# Autodesk Inventor assembly: rigt_motor_asembly
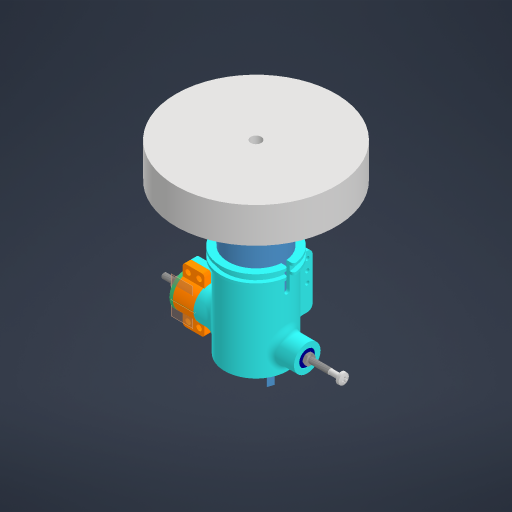
[picture p0: Inventor's stored thumbnail of the model, 512x512]
Saved by Autodesk Inventor 2024 (Build 280153000, 153)
## iProperties
Created: 2023-05-14
Part Number: rigt_motor_asembly
Document SubType Name: Assembly
Designer: user
Author: user
## Documents named in this file (9)
- D:\Docs\Robot\3d\motor_assembly\left_motor_asembly.iam
- D:\Docs\Robot\3d\motor_assembly\bushing_assembly.iam
- D:\Docs\Robot\3d\default_components\motor.ipt
- D:\Docs\Robot\3d\default_components\wheel.ipt
- D:\Docs\Robot\3d\default_components\604zz_bearing.ipt
- C:\Users\user\Documents\Inventor\Content Center Files\R2024\ru-RU\DIN 934\DIN 934 - M4 x 0,7.ipt
- D:\Docs\Robot\3d\motor_assembly\default_motor_asembly\cup.ipt
- D:\Docs\Robot\3d\motor_assembly\left_motor_asembly\lower_arm.ipt
- C:\Users\user\Documents\Inventor\Content Center Files\R2024\ru-RU\DIN 7985 (H)\DIN 7985 (H) - M4x30-H.ipt
## Components (8 placed, 8 different names)
1. lower_arm:2 — Вставка:11, Вставка:12, Вставка:13, Вставка:14, Вставка:15
2. bushing_assembly:2 [sub-assembly] — Вставка:14
3. motor:1 — Вставка:4, Вставка:11
4. wheel:1 — Вставка:4
5. 604zz_bearing:1 — Вставка:8, Вставка:15, Вставка:16
6. DIN 934 - заменено на DIN EN 24032/28673/28674 M4:1 — Вставка:8
7. cup:1 — Вставка:12, Вставка:13
8. DIN 7985 (H) M4x30-H:1 — Вставка:16
## Relationships (12: Insert 8, Mate 4)
- [Mate]: lower_arm:2
- [Mate]: lower_arm:2
- [Mate]: lower_arm:2
- Вставка:4 [Insert]: motor:1 ↔ wheel:1
- [Mate]: lower_arm:2
- Вставка:8 [Insert]: 604zz_bearing:1 ↔ DIN 934 - заменено на DIN EN 24032/28673/28674 M4:1
- Вставка:11 [Insert]: lower_arm:2 ↔ motor:1
- Вставка:12 [Insert]: lower_arm:2 ↔ cup:1
- Вставка:13 [Insert]: lower_arm:2 ↔ cup:1
- Вставка:14 [Insert]: lower_arm:2 ↔ bushing_assembly:2
- Вставка:15 [Insert]: lower_arm:2 ↔ 604zz_bearing:1
- Вставка:16 [Insert]: 604zz_bearing:1 ↔ DIN 7985 (H) M4x30-H:1
